# Autodesk Inventor assembly: LiftPrototypeMKI
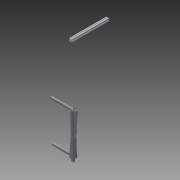
[picture p0: Inventor's stored thumbnail of the model, 180x180]
Saved by Autodesk Inventor 2013 (Build 170138000, 138)
## iProperties
Created: 2013-10-02
Part Number: LiftPrototypeMKI
Document SubType Name: Assembly
Designer: cobrooks
Author: cobrooks
## Documents named in this file (7)
- C:\Users\cobrooks\Documents\Robotics\2013-14\CAD\Lift\LiftPrototype\LiftPrototypeMKI.iam
- \\lmss\STUDENTS\Robotics\CAD Files\COTS Parts\Bosch Extrusion\Bosch 20x20.ipt
- \\lmss\STUDENTS\Robotics\CAD Files\5x5mm Box Aluminum.ipt
- \\lmss\STUDENTS\Robotics\CAD Files\COTS Parts\Fasteners\14-20 Washer - Flat.ipt
- \\lmss\STUDENTS\Robotics\CAD Files\COTS Parts\Fasteners\8-32 BHCS x1500.ipt
- \\lmss\STUDENTS\Robotics\CAD Files\COTS Parts\Fasteners\8-32 locknut.ipt
- \\lmss\STUDENTS\Robotics\CAD Files\ShortBox.ipt
## Components (25 placed, 6 different names)
1. Bosch 20x20:1
2. 14-20 Washer - Flat:1 — Insert:2, Insert:3
3. 5x5mm Box Aluminum:1 — Insert:1, Insert:2, Insert:12, Insert:15, Insert:20, Insert:23
4. 5x5mm Box Aluminum:2 — Insert:3, Insert:4, Insert:11, Insert:16, Insert:18, Insert:22
5. 8-32 BHCS x1500:1 — Insert:1
6. 8-32 locknut:1 — Insert:4
7. 5x5mm Box Aluminum:3 — Insert:5, Insert:6, Insert:9, Insert:13
8. 5x5mm Box Aluminum:4 — Insert:7, Insert:8, Insert:10, Insert:14
9. 8-32 BHCS x1500:2 — Insert:5
10. 8-32 locknut:2 — Insert:8
11. 14-20 Washer - Flat:3 — Insert:6, Insert:7
12. 14-20 Washer - Flat:4 — Insert:17, Insert:18
13. 8-32 BHCS x1500:3 — Insert:21
14. 8-32 locknut:3 — Insert:22
15. 14-20 Washer - Flat:5 — Insert:9, Insert:12
16. 14-20 Washer - Flat:6 — Insert:10, Insert:11
17. 8-32 BHCS x1500:4 — Insert:13
18. 8-32 BHCS x1500:5 — Insert:14
19. 8-32 locknut:4 — Insert:15
20. 8-32 locknut:5 — Insert:16
21. ShortBox:1 — Insert:17, Insert:21
22. ShortBox:2 — Insert:19, Insert:24
23. 14-20 Washer - Flat:7 — Insert:19, Insert:20
24. 8-32 locknut:6 — Insert:24
25. 8-32 BHCS x1500:6 — Insert:23
## Relationships (24: Insert 24)
- Insert:1: 5x5mm Box Aluminum:1 ↔ 8-32 BHCS x1500:1
- Insert:2: 14-20 Washer - Flat:1 ↔ 5x5mm Box Aluminum:1
- Insert:3: 14-20 Washer - Flat:1 ↔ 5x5mm Box Aluminum:2
- Insert:4: 5x5mm Box Aluminum:2 ↔ 8-32 locknut:1
- Insert:5: 5x5mm Box Aluminum:3 ↔ 8-32 BHCS x1500:2
- Insert:6: 5x5mm Box Aluminum:3 ↔ 14-20 Washer - Flat:3
- Insert:7: 5x5mm Box Aluminum:4 ↔ 14-20 Washer - Flat:3
- Insert:8: 5x5mm Box Aluminum:4 ↔ 8-32 locknut:2
- Insert:9: 5x5mm Box Aluminum:3 ↔ 14-20 Washer - Flat:5
- Insert:10: 5x5mm Box Aluminum:4 ↔ 14-20 Washer - Flat:6
- Insert:11: 5x5mm Box Aluminum:2 ↔ 14-20 Washer - Flat:6
- Insert:12: 5x5mm Box Aluminum:1 ↔ 14-20 Washer - Flat:5
- Insert:13: 5x5mm Box Aluminum:3 ↔ 8-32 BHCS x1500:4
- Insert:14: 5x5mm Box Aluminum:4 ↔ 8-32 BHCS x1500:5
- Insert:15: 5x5mm Box Aluminum:1 ↔ 8-32 locknut:4
- Insert:16: 5x5mm Box Aluminum:2 ↔ 8-32 locknut:5
- Insert:17: 14-20 Washer - Flat:4 ↔ ShortBox:1
- Insert:18: 5x5mm Box Aluminum:2 ↔ 14-20 Washer - Flat:4
- Insert:19: ShortBox:2 ↔ 14-20 Washer - Flat:7
- Insert:20: 5x5mm Box Aluminum:1 ↔ 14-20 Washer - Flat:7
- Insert:21: 8-32 BHCS x1500:3 ↔ ShortBox:1
- Insert:22: 5x5mm Box Aluminum:2 ↔ 8-32 locknut:3
- Insert:23: 5x5mm Box Aluminum:1 ↔ 8-32 BHCS x1500:6
- Insert:24: ShortBox:2 ↔ 8-32 locknut:6
